# Autodesk Inventor assembly: Сборка2
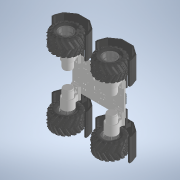
[picture p0: Inventor's stored thumbnail of the model, 180x180]
Saved by Autodesk Inventor 2022 (Build 260153000, 153)
## iProperties
Created: 2023-05-17
Part Number: Сборка2
Document SubType Name: Assembly
Designer: korsh624
Author: korsh624
## Documents named in this file (6)
- C:\git\robot_01\design\Сборка2.iam
- C:\git\robot_01\design\драйвер.ipt
- C:\git\robot_01\design\MEGA 2560 PRO (EMBED).iam
- C:\git\robot_01\design\motor_krilo.iam
- C:\git\robot_01\design\base.ipt
- C:\git\robot_01\design\Сборка13.iam
## Components (9 placed, 5 different names)
1. motor_krilo:1 [sub-assembly] — Заподлицо:12, Заподлицо:13, Совмещение:4, Заподлицо:16, Совмещение:6, Совмещение:8
2. motor_krilo:2 [sub-assembly] — Заподлицо:12, Заподлицо:13, Совмещение:4, Заподлицо:17, Заподлицо:20
3. motor_krilo:3 [sub-assembly] — Заподлицо:14, Заподлицо:15, Совмещение:5, Заподлицо:16, Заподлицо:17
4. motor_krilo:4 [sub-assembly] — Заподлицо:14, Заподлицо:15, Совмещение:5, Совмещение:6
5. base:1 — Заподлицо:20, Совмещение:7, Заподлицо:21, Совмещение:9, Совмещение:11, Заподлицо:24, Заподлицо:25
6. MEGA 2560 PRO (EMBED):1 [sub-assembly] — Совмещение:7, Заподлицо:21, Совмещение:8
7. драйвер:1 — Заподлицо:22, Совмещение:10, Заподлицо:23
8. драйвер:2 — Заподлицо:22, Совмещение:9, Совмещение:10, Заподлицо:23
9. Сборка13:1 [sub-assembly] — Совмещение:11, Заподлицо:24, Заподлицо:25
## Relationships (20: Flush 12, Mate 8)
- Заподлицо:12 [Flush]: motor_krilo:1 ↔ motor_krilo:2
- Заподлицо:13 [Flush]: motor_krilo:1 ↔ motor_krilo:2
- Заподлицо:14 [Flush]: motor_krilo:3 ↔ motor_krilo:4
- Заподлицо:15 [Flush]: motor_krilo:3 ↔ motor_krilo:4
- Совмещение:4 [Mate] (150 mm): motor_krilo:1 ↔ motor_krilo:2
- Совмещение:5 [Mate] (150 mm): motor_krilo:3 ↔ motor_krilo:4
- Заподлицо:16 [Flush]: motor_krilo:1 ↔ motor_krilo:3
- Совмещение:6 [Mate] (80 mm): motor_krilo:1 ↔ motor_krilo:4
- Заподлицо:17 [Flush]: motor_krilo:2 ↔ motor_krilo:3
- Заподлицо:20 [Flush]: motor_krilo:2 ↔ base:1
- Совмещение:7 [Mate]: base:1 ↔ MEGA 2560 PRO (EMBED):1
- Заподлицо:21 [Flush]: base:1 ↔ MEGA 2560 PRO (EMBED):1
- Совмещение:8 [Mate] (20 mm): motor_krilo:1 ↔ MEGA 2560 PRO (EMBED):1
- Заподлицо:22 [Flush]: драйвер:1 ↔ драйвер:2
- Совмещение:9 [Mate]: base:1 ↔ драйвер:2
- Совмещение:10 [Mate] (40 mm): драйвер:1 ↔ драйвер:2
- Заподлицо:23 [Flush]: драйвер:1 ↔ драйвер:2
- Совмещение:11 [Mate]: base:1 ↔ Сборка13:1
- Заподлицо:24 [Flush]: base:1 ↔ Сборка13:1
- Заподлицо:25 [Flush]: base:1 ↔ Сборка13:1
